# Autodesk Inventor assembly: V3LeftClimbTower
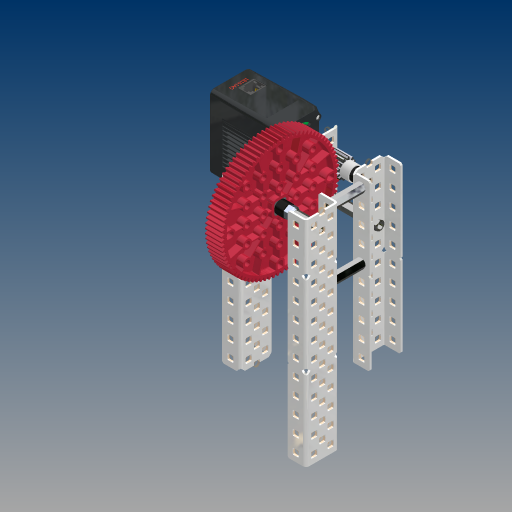
[picture p0: Inventor's stored thumbnail of the model, 512x512]
Saved by Autodesk Inventor 2023 (Build 270158000, 158)
## iProperties
Created: 2023-10-21
Part Number: V3LeftClimbTower
Document SubType Name: Assembly
Designer: eddie
Author: eddie
## Documents named in this file (20)
- C:\Users\eddie\Documents\81208X-Over-Under-CAD\V3\V3LeftClimbTower.iam
- C:\Users\eddie\Documents\81208X-Over-Under-CAD\VEX-CAD-Inventor-1.4.0\Structure\C Channel\Aluminum 1x2x1\Alu C 1x2x1x13.ipt
- C:\Users\eddie\Documents\81208X-Over-Under-CAD\VEX-CAD-Inventor-1.4.0\Structure\Standoff\Standoff .75.ipt
- C:\Users\eddie\Documents\81208X-Over-Under-CAD\VEX-CAD-Inventor-1.4.0\Structure\Standoff.ipt
- C:\Users\eddie\Documents\81208X-Over-Under-CAD\VEX-CAD-Inventor-1.4.0\Structure\Hardware\Nut Nylock.ipt
- C:\Users\eddie\Documents\81208X-Over-Under-CAD\VEX-CAD-Inventor-1.4.0\Motion\Spacers\Spacer Nylon .375 OD\NSpacer .375 OD x .250.ipt
- C:\Users\eddie\Documents\81208X-Over-Under-CAD\VEX-CAD-Inventor-1.4.0\Motion\Spacers\Spacer Nylon .375 OD.ipt
- C:\Users\eddie\Documents\81208X-Over-Under-CAD\VEX-CAD-Inventor-1.4.0\Motion\Gears\HS Gear.iam
- C:\Users\eddie\Documents\81208X-Over-Under-CAD\VEX-CAD-Inventor-1.4.0\Motion\Spacers\Washer Steel\SWasher .375 OD x .031250.ipt
- C:\Users\eddie\Documents\81208X-Over-Under-CAD\VEX-CAD-Inventor-1.4.0\Motion\Spacers\Washer Steel.ipt
- C:\Users\eddie\Documents\81208X-Over-Under-CAD\VEX-CAD-Inventor-1.4.0\Structure\Hardware\Nut Keps.ipt
- C:\Users\eddie\Documents\81208X-Over-Under-CAD\VEX-CAD-Inventor-1.4.0\Structure\C Channel\Aluminum 1x2x1\Alu C 1x2x1x10.ipt
- C:\Users\eddie\Documents\81208X-Over-Under-CAD\VEX-CAD-Inventor-1.4.0\Structure\Standoff\Standoff 1.00.ipt
- C:\Users\eddie\Documents\81208X-Over-Under-CAD\Custom-parts\2x4 channel without 1 side.ipt
- C:\Users\eddie\Documents\81208X-Over-Under-CAD\VEX-CAD-Inventor-1.4.0\Motion\Spacers\Spacer Nylon .375 OD\NSpacer .375 OD x .375.ipt
- C:\Users\eddie\Documents\81208X-Over-Under-CAD\Custom-parts\Shaft Collar.ipt
- C:\Users\eddie\Documents\81208X-Over-Under-CAD\VEX-CAD-Inventor-1.4.0\Motion\Gears\HS Gear\HS 12T Gear, Square.iam
- C:\Users\eddie\Documents\81208X-Over-Under-CAD\VEX-CAD-Inventor-1.4.0\Motion\Gears\HS Gear\HS 84T Gear, Circle.iam
- C:\Users\eddie\Documents\81208X-Over-Under-CAD\VEX-CAD-Inventor-1.4.0\Structure\Standoff\Standoff 1.50.ipt
- C:\Users\eddie\Documents\81208X-Over-Under-CAD\VEX-CAD-Inventor-1.4.0\Electronics\V5 Motor.ipt
## Components (21 placed, 15 different names)
1. Alu C 1x2x1x13:1 — Insert:1, Insert:9, Insert:19
2. Standoff .75:1 — Insert:1, Insert:2
3. Nut Nylock:1 — Insert:2, Insert:3
4. NSpacer .375 OD x .250:1 — Insert:3, Insert:17
5. SWasher .375 OD x .031250:1 — Insert:6
6. SWasher .375 OD x .031250:2 — Insert:6, Insert:7
7. Nut Keps:1 — Insert:7, Insert:8
8. Alu C 1x2x1x10:1 — Insert:8, Insert:10
9. Standoff 1.00:2 — Insert:10, Insert:12
10. Standoff 1.00:3 — Insert:9, Insert:11
11. Alu C 1x2x1x10:2 — Insert:11, Insert:13
12. 2x4 channel without 1 side:1 — Insert:12, Insert:18, Insert:20, Insert:21
13. NSpacer .375 OD x .375:2 — Insert:13, Insert:14
14. Shaft Collar:1 — Insert:14, Insert:15
15. HS 12T Gear, Square:2 [sub-assembly] — Insert:15, Insert:16
16. NSpacer .375 OD x .250:3 — Insert:16
17. HS 84T Gear, Circle:3 [sub-assembly] — Insert:17
18. Standoff 1.50:4 — Insert:18
19. Standoff 1.00:5 — Insert:19
20. Standoff 1.00:6 — Insert:20
21. V5 Motor:1 — Insert:21
## Relationships (19: Insert 19)
- Insert:1: Alu C 1x2x1x13:1 ↔ Standoff .75:1
- Insert:2: Standoff .75:1 ↔ Nut Nylock:1
- Insert:3: Nut Nylock:1 ↔ NSpacer .375 OD x .250:1
- Insert:6: SWasher .375 OD x .031250:1 ↔ SWasher .375 OD x .031250:2
- Insert:7: SWasher .375 OD x .031250:2 ↔ Nut Keps:1
- Insert:8: Nut Keps:1 ↔ Alu C 1x2x1x10:1
- Insert:9: Alu C 1x2x1x13:1 ↔ Standoff 1.00:3
- Insert:10: Alu C 1x2x1x10:1 ↔ Standoff 1.00:2
- Insert:11: Standoff 1.00:3 ↔ Alu C 1x2x1x10:2
- Insert:12: Standoff 1.00:2 ↔ 2x4 channel without 1 side:1
- Insert:13: Alu C 1x2x1x10:2 ↔ NSpacer .375 OD x .375:2
- Insert:14: NSpacer .375 OD x .375:2 ↔ Shaft Collar:1
- Insert:15: Shaft Collar:1 ↔ HS 12T Gear, Square:2
- Insert:16: HS 12T Gear, Square:2 ↔ NSpacer .375 OD x .250:3
- Insert:17: NSpacer .375 OD x .250:1 ↔ HS 84T Gear, Circle:3
- Insert:18: 2x4 channel without 1 side:1 ↔ Standoff 1.50:4
- Insert:19: Alu C 1x2x1x13:1 ↔ Standoff 1.00:5
- Insert:20: 2x4 channel without 1 side:1 ↔ Standoff 1.00:6
- Insert:21: 2x4 channel without 1 side:1 ↔ V5 Motor:1
